# Autodesk Inventor assembly: filterMount
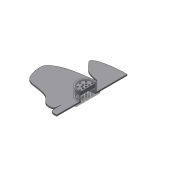
[picture p0: Inventor's stored thumbnail of the model, 180x180]
Saved by Autodesk Inventor 2018 (Build 220112000, 112)
## iProperties
Created: 2020-03-26
Part Number: filterMount
Document SubType Name: Assembly
Designer: Matt
Author: Matt
## Documents named in this file (5)
- C:\Users\Matt\n95\filterMount.iam
- C:\Users\Matt\n95\insideFlange.ipt
- C:\Users\Matt\n95\middleFlange.ipt
- C:\Users\Matt\n95\lid.ipt
- C:\Users\Matt\n95\rubberFlatPatternSheetMetal.ipt
## Components (4 placed, 4 different names)
1. insideFlange:1 — Flush:1, Flush:2, Mate:1
2. middleFlange:1 — Flush:1
3. lid:1 — Flush:2
4. rubberFlatPatternSheetMetal:1 — Mate:1
## Relationships (3: Flush 2, Mate 1)
- Flush:1 (2.3813 mm): insideFlange:1 ↔ middleFlange:1
- Flush:2 (3.175 mm): insideFlange:1 ↔ lid:1
- Mate:1: insideFlange:1 ↔ rubberFlatPatternSheetMetal:1
